# Autodesk Inventor assembly: V-Belt transmission
Saved by Autodesk Inventor 2014 SP1 (Build 180222100, 222)
## iProperties
Created: 2014-01-12
Part Number: V-Belt transmission
Document SubType Name: Assembly
Designer: Ryan
ClientObjectVersion: 1
Author: Ryan
## Documents named in this file (3)
- C:\Users\Ryan\Desktop\sw\toss up 1st A bot\inventor drive\manual shifter\Design Accelerator\V-Belt transmission2.iam
- C:\Users\Ryan\Desktop\sw\toss up 1st A bot\inventor drive\manual shifter\Design Accelerator\V-Belt2.ipt
- C:\Users\Ryan\Desktop\sw\toss up 1st A bot\inventor drive\manual shifter\Design Accelerator\Flat Pulley31.ipt
## Components (2 placed, 2 different names)
1. Flat Pulley3:1 — Flush:1, Mate:1
2. V-Belt:1 — Flush:1, Mate:1
## Component patterns: (1 elements, first: V-Belt:1)
## Relationships (2: Flush 1, Mate 1)
- Flush:1: Flat Pulley3:1 ↔ V-Belt:1
- Mate:1: Flat Pulley3:1 ↔ V-Belt:1
